# Autodesk Inventor assembly: controller
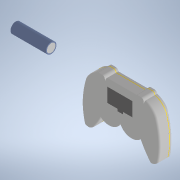
[picture p0: Inventor's stored thumbnail of the model, 180x180]
Saved by Autodesk Inventor 2022 (Build 260153000, 153)
## iProperties
Created: 2022-12-06
Part Number: controller
Document SubType Name: Assembly
Designer: matys
Author: matys
## Documents named in this file (6)
- C:\Users\matys\Desktop\remote-controller\inventor\controller.iam
- C:\Users\matys\Desktop\Práce4tak\Inventor\hardware_modules\baterka.ipt
- C:\Users\matys\Desktop\remote-controller\inventor\ovladac.ipt
- C:\Users\matys\Desktop\remote-controller\inventor\ovladac - dole.ipt
- C:\Users\matys\Desktop\remote-controller\inventor\ovladac - nahore.ipt
- C:\Users\matys\Desktop\remote-controller\inventor\poklop.ipt
## Components (5 placed, 5 different names)
1. baterka:1
2. ovladac:1 — Mate:1, Mate:2, Mate:3, Mate:4
3. ovladac - dole:1 — Mate:1, Mate:2, Mate:5, Mate:6
4. ovladac - nahore:2 — Mate:3, Mate:4
5. poklop:1 — Mate:5, Mate:6
## Relationships (6: Mate 6)
- Mate:1: ovladac:1 ↔ ovladac - dole:1
- Mate:2: ovladac:1 ↔ ovladac - dole:1
- Mate:3: ovladac:1 ↔ ovladac - nahore:2
- Mate:4: ovladac:1 ↔ ovladac - nahore:2
- Mate:5: ovladac - dole:1 ↔ poklop:1
- Mate:6: ovladac - dole:1 ↔ poklop:1
